# Autodesk Inventor assembly: Assembly1
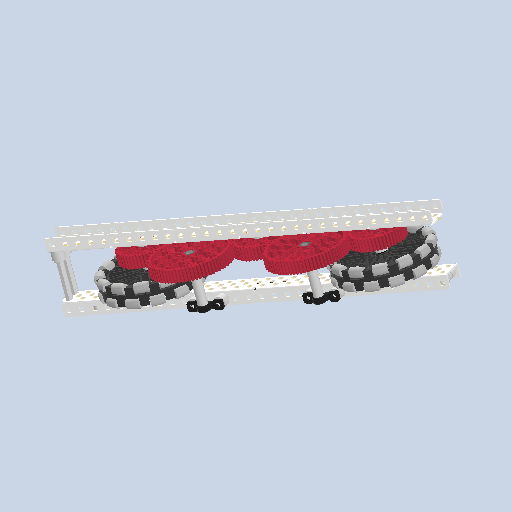
[picture p0: Inventor's stored thumbnail of the model, 512x512]
Saved by Autodesk Inventor 2024 (Build 280153000, 153)
## iProperties
Created: 2023-09-19
Part Number: Assembly1
Document SubType Name: Assembly
Designer: Robodox
Author: Robodox
## Documents named in this file (17)
- C:\Users\Robodox\Documents\GitHub\VEXCAD\Assembly1.iam
- C:\Users\Robodox\Documents\GitHub\VEX-CAD-Inventor\Structure\C Channel\Aluminum 1x2x1\Alu C 1x2x1x30.ipt
- C:\Users\Robodox\Documents\GitHub\VEX-CAD-Inventor\Motion\Gears\HS Gear.iam
- C:\Users\Robodox\Documents\GitHub\VEXCAD\Part1.ipt
- C:\Users\Robodox\Documents\GitHub\VEXCAD\Part2.ipt
- C:\Users\Robodox\Documents\GitHub\VEXCAD\Part3.ipt
- C:\Users\Robodox\Documents\GitHub\VEXCAD\Part4.ipt
- C:\Users\Robodox\Documents\GitHub\VEXCAD\Part5.ipt
- C:\Users\Robodox\Documents\GitHub\VEXCAD\part8.ipt
- C:\Users\Robodox\Documents\GitHub\VEX-CAD-Inventor\Motion\Wheels\Omni Wheel\4 Omni AS, Square.iam
- C:\Users\Robodox\Documents\GitHub\VEX-CAD-Inventor\Motion\Wheels\Omni Wheel.iam
- C:\Users\Robodox\Documents\GitHub\VEX-CAD-Inventor\Motion\Gears\HS Gear\HS 72T Gear, Square.iam
- C:\Users\Robodox\Documents\GitHub\VEX-CAD-Inventor\Motion\Gears\HS Gear\HS 48T Gear, Square.iam
- C:\Users\Robodox\Documents\GitHub\VEX-CAD-Inventor\Motion\Shaft LS\Bearing Flat.ipt
- C:\Users\Robodox\Documents\GitHub\VEX-CAD-Inventor\Motion\Shaft LS\LS Pillow Bearing Block.ipt
- C:\Users\Robodox\Documents\GitHub\VEX-CAD-Inventor\Motion\Shaft LS\Shaft Collar ipts\Shaft Collar Set Screw.ipt
- C:\Users\Robodox\Documents\GitHub\VEXCAD\washer.ipt
## Components (57 placed, 14 different names)
1. Alu C 1x2x1x30:1 — Flush:1, Flush:2, Mate:1, Mate:2, Mate:7, Mate:11, Mate:12, Mate:15, Mate:27, Mate:31, Mate:32, Mate:33, Mate:34, Mate:35, Mate:36, Mate:37, Mate:38, Mate:110, Mate:111, Mate:112, Mate:113, Mate:114, Mate:115, Mate:116, Mate:117, Mate:118, Mate:119, Mate:120, Mate:167, Mate:170, Flush:3, Mate:175, Mate:176
2. Alu C 1x2x1x30:2 — Flush:1, Flush:2, Mate:20, Mate:74, Flush:3, Mate:175, Mate:176
3. Part2:5 — Mate:13, Mate:14, Mate:28, Mate:29
4. Part1:9 — Mate:14, Mate:29
5. Part1:10 — Mate:12, Mate:13, Mate:15, Mate:28
6. Part3:3 — Mate:31, Mate:32, Mate:121, Mate:125
7. Part3:4 — Mate:33, Mate:38, Mate:126
8. Part3:5 — Mate:34, Mate:37, Mate:122, Mate:123
9. Part3:6 — Mate:35, Mate:36, Mate:124
10. Part5:1 — Mate:47, Mate:52, Mate:128, Mate:154
11. Part5:2 — Mate:48, Mate:49, Mate:127, Mate:156
12. Part5:3 — Mate:47, Mate:52, Mate:152, Mate:153
13. Part5:4 — Mate:48, Mate:49, Mate:151, Mate:155
14. part8:1 — Mate:132, Mate:158, Mate:173
15. part8:2 — Mate:159, Mate:160, Mate:174
16. part8:3 — Mate:74, Mate:131, Mate:133, Mate:150, Mate:157
17. Part3:11 — Mate:90, Mate:129, Mate:161, Mate:162
18. Part3:12 — Mate:87, Mate:130, Mate:134, Mate:163
19. 4 Omni AS, Square:1 [sub-assembly] — Mate:87, Mate:137, Mate:138, Mate:163
20. 4 Omni AS, Square:2 [sub-assembly] — Mate:90, Mate:142, Mate:143, Mate:162
21. Bearing Flat:3 — Mate:118, Mate:119, Mate:120, Mate:159
22. Bearing Flat:4 — Mate:115, Mate:116, Mate:117, Mate:157
23. Bearing Flat:5 — Mate:112, Mate:113, Mate:114, Mate:158
24. LS Pillow Bearing Block:1 — Mate:122, Mate:123, Mate:124, Mate:152, Mate:153
25. LS Pillow Bearing Block:2 — Mate:121, Mate:125, Mate:126, Mate:151, Mate:155
26. HS 72T Gear, Square:1 [sub-assembly] — Mate:127, Mate:156
27. HS 72T Gear, Square:2 [sub-assembly] — Mate:128, Mate:154
28. HS 48T Gear, Square:3 [sub-assembly] — Mate:131, Mate:133, Mate:148, Mate:149
29. HS 48T Gear, Square:4 [sub-assembly] — Mate:130, Mate:134, Mate:160, Mate:174
30. HS 48T Gear, Square:5 [sub-assembly] — Mate:129, Mate:132, Mate:161, Mate:173
31. Shaft Collar Set Screw:1 — Mate:137, Mate:138, Mate:168, Mate:169
32. Shaft Collar Set Screw:2 — Mate:142, Mate:143, Mate:171, Mate:172
33. Shaft Collar Set Screw:3 — Mate:148, Mate:149, Mate:150
34. washer:3 — Mate:167, Mate:168, Mate:169
35. washer:4 — Mate:170, Mate:171, Mate:172
36. Part1:1 — Mate:4, Mate:5
37. Part2:1 — Mate:3, Mate:4, Mate:5, Mate:6
38. Part1:2 — Mate:1, Mate:2, Mate:3, Mate:6
39. Part1:3
40. Part2:2
41. Part1:4
42. Part1:6 — Mate:9, Mate:10
43. Part2:3 — Mate:8, Mate:9, Mate:10, Mate:30
44. Part1:5 — Mate:7, Mate:8, Mate:11, Mate:30
45. Part1:7
46. Part2:4
47. Part1:8
48. Part1:12 — Mate:108, Mate:109, Mate:110, Mate:111
49. Part2:7 — Mate:108, Mate:109
50. Part1:13
51. Part2:8
52. Part3:1 — Mate:20, Mate:25, Mate:164, Mate:165
53. washer:1 — Mate:164, Mate:165, Mate:166
54. Part4:1 — Mate:25, Mate:27, Mate:166
55. Part3:13
56. washer:2
57. Part4:2
## Component patterns: (2 elements, first: Part1:1 + Part2:1 + Part1:2), (2 elements, first: Part1:6 + Part2:3 + Part1:5), (2 elements, first: Part1:12 + Part2:7), (2 elements, first: Part3:1 + washer:1 + Part4:1)
## Relationships (99: Mate 96, Flush 3)
- Flush:1: Alu C 1x2x1x30:1 ↔ Alu C 1x2x1x30:2
- Flush:2: Alu C 1x2x1x30:1 ↔ Alu C 1x2x1x30:2
- Mate:1: Alu C 1x2x1x30:1 ↔ Part1:2
- Mate:2: Alu C 1x2x1x30:1 ↔ Part1:2
- Mate:3: Part2:1 ↔ Part1:2
- Mate:4: Part1:1 ↔ Part2:1
- Mate:5: Part1:1 ↔ Part2:1
- Mate:6: Part2:1 ↔ Part1:2
- Mate:7: Alu C 1x2x1x30:1 ↔ Part1:5
- Mate:8: Part2:3 ↔ Part1:5
- Mate:9: Part1:6 ↔ Part2:3
- Mate:10: Part1:6 ↔ Part2:3
- Mate:11: Alu C 1x2x1x30:1 ↔ Part1:5
- Mate:12: Alu C 1x2x1x30:1 ↔ Part1:10
- Mate:13: Part2:5 ↔ Part1:10
- Mate:14: Part2:5 ↔ Part1:9
- Mate:15: Alu C 1x2x1x30:1 ↔ Part1:10
- Mate:20: Alu C 1x2x1x30:2 ↔ Part3:1
- Mate:25: Part3:1 ↔ Part4:1
- Mate:27: Alu C 1x2x1x30:1 ↔ Part4:1
- Mate:28: Part2:5 ↔ Part1:10
- Mate:29: Part2:5 ↔ Part1:9
- Mate:30: Part2:3 ↔ Part1:5
- Mate:31: Alu C 1x2x1x30:1 ↔ Part3:3
- Mate:32: Alu C 1x2x1x30:1 ↔ Part3:3
- Mate:33: Alu C 1x2x1x30:1 ↔ Part3:4
- Mate:34: Alu C 1x2x1x30:1 ↔ Part3:5
- Mate:35: Alu C 1x2x1x30:1 ↔ Part3:6
- Mate:36: Alu C 1x2x1x30:1 ↔ Part3:6
- Mate:37: Alu C 1x2x1x30:1 ↔ Part3:5
- Mate:38: Alu C 1x2x1x30:1 ↔ Part3:4
- Mate:47: Part5:1 ↔ Part5:3
- Mate:48: Part5:2 ↔ Part5:4
- Mate:49: Part5:2 ↔ Part5:4
- Mate:52: Part5:1 ↔ Part5:3
- Mate:74: Alu C 1x2x1x30:2 ↔ part8:3
- Mate:87: Part3:12 ↔ 4 Omni AS, Square:1
- Mate:90: Part3:11 ↔ 4 Omni AS, Square:2
- Mate:108: Part1:12 ↔ Part2:7
- Mate:109: Part1:12 ↔ Part2:7
- Mate:110: Alu C 1x2x1x30:1 ↔ Part1:12
- Mate:111: Alu C 1x2x1x30:1 ↔ Part1:12
- Mate:112: Alu C 1x2x1x30:1 ↔ Bearing Flat:5
- Mate:113: Alu C 1x2x1x30:1 ↔ Bearing Flat:5
- Mate:114: Alu C 1x2x1x30:1 ↔ Bearing Flat:5
- Mate:115: Alu C 1x2x1x30:1 ↔ Bearing Flat:4
- Mate:116: Alu C 1x2x1x30:1 ↔ Bearing Flat:4
- Mate:117: Alu C 1x2x1x30:1 ↔ Bearing Flat:4
- Mate:118: Alu C 1x2x1x30:1 ↔ Bearing Flat:3
- Mate:119: Alu C 1x2x1x30:1 ↔ Bearing Flat:3
- Mate:120: Alu C 1x2x1x30:1 ↔ Bearing Flat:3
- Mate:121: Part3:3 ↔ LS Pillow Bearing Block:2
- Mate:122: Part3:5 ↔ LS Pillow Bearing Block:1
- Mate:123: Part3:5 ↔ LS Pillow Bearing Block:1
- Mate:124: Part3:6 ↔ LS Pillow Bearing Block:1
- Mate:125: Part3:3 ↔ LS Pillow Bearing Block:2
- Mate:126: Part3:4 ↔ LS Pillow Bearing Block:2
- Mate:127: Part5:2 ↔ HS 72T Gear, Square:1
- Mate:128: Part5:1 ↔ HS 72T Gear, Square:2
- Mate:129: Part3:11 ↔ HS 48T Gear, Square:5
- Mate:130: Part3:12 ↔ HS 48T Gear, Square:4
- Mate:131: part8:3 ↔ HS 48T Gear, Square:3
- Mate:132: part8:1 ↔ HS 48T Gear, Square:5
- Mate:133: part8:3 ↔ HS 48T Gear, Square:3
- Mate:134: Part3:12 ↔ HS 48T Gear, Square:4
- Mate:137: 4 Omni AS, Square:1 ↔ Shaft Collar Set Screw:1
- Mate:138: 4 Omni AS, Square:1 ↔ Shaft Collar Set Screw:1
- Mate:142: 4 Omni AS, Square:2 ↔ Shaft Collar Set Screw:2
- Mate:143: 4 Omni AS, Square:2 ↔ Shaft Collar Set Screw:2
- Mate:148: HS 48T Gear, Square:3 ↔ Shaft Collar Set Screw:3
- Mate:149: HS 48T Gear, Square:3 ↔ Shaft Collar Set Screw:3
- Mate:150: part8:3 ↔ Shaft Collar Set Screw:3
- Mate:151: Part5:4 ↔ LS Pillow Bearing Block:2
- Mate:152: Part5:3 ↔ LS Pillow Bearing Block:1
- Mate:153: Part5:3 ↔ LS Pillow Bearing Block:1
- Mate:154: Part5:1 ↔ HS 72T Gear, Square:2
- Mate:155: Part5:4 ↔ LS Pillow Bearing Block:2
- Mate:156: Part5:2 ↔ HS 72T Gear, Square:1
- Mate:157: part8:3 ↔ Bearing Flat:4
- Mate:158: part8:1 ↔ Bearing Flat:5
- Mate:159: part8:2 ↔ Bearing Flat:3
- Mate:160: part8:2 ↔ HS 48T Gear, Square:4
- Mate:161: Part3:11 ↔ HS 48T Gear, Square:5
- Mate:162: Part3:11 ↔ 4 Omni AS, Square:2
- Mate:163: Part3:12 ↔ 4 Omni AS, Square:1
- Mate:164: Part3:1 ↔ washer:1
- Mate:165: Part3:1 ↔ washer:1
- Mate:166: washer:1 ↔ Part4:1
- Mate:167: Alu C 1x2x1x30:1 ↔ washer:3
- Mate:168: Shaft Collar Set Screw:1 ↔ washer:3
- Mate:169: Shaft Collar Set Screw:1 ↔ washer:3
- Mate:170: Alu C 1x2x1x30:1 ↔ washer:4
- Mate:171: Shaft Collar Set Screw:2 ↔ washer:4
- Mate:172: Shaft Collar Set Screw:2 ↔ washer:4
- Flush:3: Alu C 1x2x1x30:1 ↔ Alu C 1x2x1x30:2
- Mate:173: part8:1 ↔ HS 48T Gear, Square:5
- Mate:174: part8:2 ↔ HS 48T Gear, Square:4
- Mate:175 (63.5 mm): Alu C 1x2x1x30:1 ↔ Alu C 1x2x1x30:2
- Mate:176 (63.5 mm): Alu C 1x2x1x30:1 ↔ Alu C 1x2x1x30:2
